# Autodesk Inventor assembly: frame
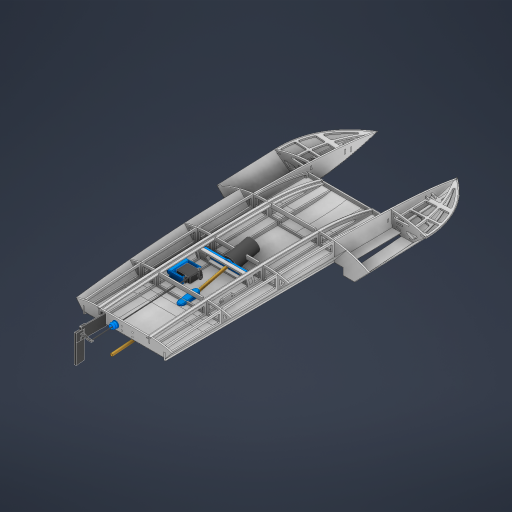
[picture p0: Inventor's stored thumbnail of the model, 512x512]
Saved by Autodesk Inventor 2023 (Build 270158030, 158C)
## iProperties
Created: 2022-03-21
Part Number: frame
Document SubType Name: Assembly
Designer: kardo
Mass: 464.87 g
Surface Area: 7011.93 cm^2
Volume: 464.87 cm^3
Density: 1 g/cm^3
Author: kardo
## Documents named in this file (42)
- D:\Computer Aided Design\hydroplane_plan_2_refactor\model\shape\frame\frame.iam
- D:\Computer Aided Design\hydroplane_plan_2_refactor\model\shape\frame\bulkheads\main.ipt
- D:\Computer Aided Design\hydroplane_plan_2_refactor\model\shape\frame\bulkheads\transom.ipt
- D:\Computer Aided Design\hydroplane_plan_2_refactor\model\shape\frame\bulkheads\stringer.ipt
- D:\Computer Aided Design\hydroplane_plan_2_refactor\model\shape\frame\bulkheads\tail_2.ipt
- D:\Computer Aided Design\hydroplane_plan_2_refactor\model\shape\frame\bulkheads\tail_1.ipt
- D:\Computer Aided Design\hydroplane_plan_2_refactor\model\shape\frame\bulkheads\sponson_break.ipt
- D:\Computer Aided Design\hydroplane_plan_2_refactor\model\shape\frame\bulkheads\nose.ipt
- D:\Computer Aided Design\hydroplane_plan_2_refactor\model\shape\frame\bulkheads\sponson_spanner_side.ipt
- D:\Computer Aided Design\hydroplane_plan_2_refactor\model\shape\frame\bulkheads\sponson_spanner_bottom.ipt
- D:\Computer Aided Design\hydroplane_plan_2_refactor\model\shape\frame\bulkheads\sponson_spanner_bottom_holder.ipt
- D:\Computer Aided Design\hydroplane_plan_2_refactor\model\shape\frame\bulkheads\sponson_spanner_side_holder.ipt
- D:\Computer Aided Design\hydroplane_plan_2_refactor\model\shape\frame\bulkheads\stringer_cowl.ipt
- D:\Computer Aided Design\hydroplane_plan_2_refactor\model\shape\frame\bulkheads\standoff.ipt
- D:\Computer Aided Design\hydroplane_plan_2_refactor\model\shape\frame\shell\bottom.ipt
- D:\Computer Aided Design\hydroplane_plan_2_refactor\model\shape\frame\mirrored\bottom_MIR.ipt
- D:\Computer Aided Design\hydroplane_plan_2_refactor\model\shape\frame\shell\bottom_standoff.ipt
- D:\Computer Aided Design\hydroplane_plan_2_refactor\model\shape\frame\shell\sponson_bottom.ipt
- D:\Computer Aided Design\hydroplane_plan_2_refactor\model\shape\frame\mirrored\sponson_bottom_MIR.ipt
- D:\Computer Aided Design\hydroplane_plan_2_refactor\model\shape\frame\shell\sponson_indent.ipt
- D:\Computer Aided Design\hydroplane_plan_2_refactor\model\shape\frame\mirrored\sponson_indent_MIR.ipt
- D:\Computer Aided Design\hydroplane_plan_2_refactor\model\shape\frame\shell\sponson_side.ipt
- D:\Computer Aided Design\hydroplane_plan_2_refactor\model\shape\frame\mirrored\sponson_side_MIR.ipt
- D:\Computer Aided Design\hydroplane_plan_2_refactor\model\shape\frame\shell\tail_side.ipt
- D:\Computer Aided Design\hydroplane_plan_2_refactor\model\shape\frame\mirrored\tail_side_MIR.ipt
- D:\Computer Aided Design\hydroplane_plan_2_refactor\model\shape\frame\shell\cowl_liner.ipt
- D:\Computer Aided Design\hydroplane_plan_2_refactor\model\shape\frame\shell\sealing_liner.ipt
- D:\Computer Aided Design\hydroplane_plan_2_refactor\model\shape\frame\bulkheads\motor_mount.ipt
- D:\Computer Aided Design\hydroplane_plan_2_refactor\model\shape\frame\plastics\shaft_outlet.ipt
- D:\Computer Aided Design\hydroplane_plan_2_refactor\model\shape\frame\plastics\servo_mount.ipt
- D:\Computer Aided Design\hydroplane_plan_2_refactor\model\shape\frame\hardware\servo.iam
- D:\Computer Aided Design\hydroplane_plan_2_refactor\model\shape\frame\hardware\rudder.iam
- D:\Computer Aided Design\hydroplane_plan_2_refactor\model\shape\frame\hardware\steering_rod.ipt
- D:\Computer Aided Design\hydroplane_plan_2_refactor\model\shape\frame\plastics\motor_mount_plate.ipt
- D:\Computer Aided Design\hydroplane_plan_2_refactor\model\shape\frame\hardware\motor.ipt
- D:\Computer Aided Design\hydroplane_plan_2_refactor\model\shape\frame\hardware\prop_shaft.ipt
- D:\Computer Aided Design\hydroplane_plan_2_refactor\model\shape\frame\shell\deck.ipt
- D:\Computer Aided Design\hydroplane_plan_2_refactor\model\shape\frame\mirrored\deck_MIR.ipt
- D:\Computer Aided Design\hydroplane_plan_2_refactor\model\shape\frame\bulkheads\nose_spanner.ipt
- D:\Computer Aided Design\hydroplane_plan_2_refactor\model\shape\frame\shell\deck_nose.ipt
- D:\Computer Aided Design\hydroplane_plan_2_refactor\model\shape\frame\mirrored\deck_nose_MIR.ipt
- D:\Computer Aided Design\hydroplane_plan_2_refactor\model\shape\frame\plastics\servo_rod_outlet.ipt
## Components (52 placed, 41 different names)
1. main:1 — Mate:47, Mate:48, Mate:49, Mate:50, Mate:51, Mate:52, Mate:53, Mate:54, Mate:55, Mate:56, Mate:57, Mate:58, Mate:67, Mate:68, Mate:69, Mate:70, Mate:71, Mate:72, Mate:73, Mate:74, Mate:75, Mate:76, Mate:77, Mate:78, Mate:79, Mate:80, Mate:81, Mate:83, Mate:85, Mate:87, Mate:89, Mate:90, Mate:91, Mate:92, Mate:93, Mate:95, Mate:96, Mate:97, Mate:99, Mate:100, Mate:101, Mate:102, Mate:123, Mate:124, Mate:125, Mate:126, Mate:127, Mate:128, Mate:135, Mate:136, Mate:137, Mate:138
2. servo_rod_outlet:1 — Mate:145, Mate:146
3. nose_spanner:2 — Mate:132, Mate:133, Mate:134
4. nose_spanner:1 — Mate:129, Mate:130, Mate:131
5. motor_mount:1 — Mate:105, Mate:106, Mate:118, Mate:119, Mate:120
6. standoff:1 — Mate:85, Mate:86, Mate:87, Mate:88
7. standoff:2 — Mate:81, Mate:82, Mate:83, Mate:84
8. transom:1 — Mate:5, Mate:6, Mate:94, Mate:98, Mate:103, Mate:104, Mate:115, Mate:116, Mate:117, Mate:145, Mate:146
9. stringer:1 — Mate:13, Mate:14, Mate:29, Mate:30, Mate:31, Mate:32, Mate:34, Mate:53, Mate:54, Mate:133
10. stringer:2 — Mate:5, Mate:6, Mate:7, Mate:8, Mate:9, Mate:10, Mate:11, Mate:12, Mate:15, Mate:16, Mate:25, Mate:26, Mate:27, Mate:28, Mate:33, Mate:51, Mate:52, Mate:130
11. tail_2:1 — Mate:7, Mate:8
12. tail_1:1 — Mate:9, Mate:10, Mate:82, Mate:86
13. sponson_break:1 — Mate:11, Mate:12, Mate:17, Mate:19, Mate:20
14. sponson_break:2 — Mate:13, Mate:14, Mate:21, Mate:23, Mate:24
15. nose:1 — Mate:15, Mate:16, Mate:84, Mate:88, Mate:129, Mate:131, Mate:132, Mate:134
16. sponson_spanner_side:1 — Mate:17, Mate:33
17. sponson_spanner_side:2 — Mate:21, Mate:34
18. sponson_spanner_bottom:1 — Mate:19, Mate:20
19. sponson_spanner_bottom:2 — Mate:23, Mate:24
20. sponson_spanner_bottom_holder:1 — Mate:25, Mate:26
21. sponson_spanner_bottom_holder:2 — Mate:29, Mate:30
22. sponson_spanner_side_holder:1 — Mate:27, Mate:28
23. sponson_spanner_side_holder:2 — Mate:31, Mate:32
24. stringer_cowl:1 — Mate:57, Mate:58, Mate:105, Mate:106
25. stringer_cowl:2 — Mate:55, Mate:56, Mate:139, Mate:140, Mate:141
26. deck_nose:1 — Mate:135, Mate:136
27. deck_nose_MIR:1 — Mate:137, Mate:138
28. deck:1 — Mate:125, Mate:126
29. deck_MIR:1 — Mate:127, Mate:128
30. cowl_liner:1 — Mate:96, Mate:97, Mate:98
31. cowl_liner:2 — Mate:93, Mate:94, Mate:95
32. sealing_liner:1 — Mate:99, Mate:102, Mate:103
33. sealing_liner:2 — Mate:100, Mate:101, Mate:104
34. tail_side:1 — Mate:89, Mate:90
35. tail_side_MIR:1 — Mate:91, Mate:92
36. sponson_side:1 — Mate:77, Mate:78
37. sponson_side_MIR:1 — Mate:79, Mate:80
38. sponson_bottom:1 — Mate:69, Mate:70
39. sponson_bottom_MIR:1 — Mate:71, Mate:72
40. sponson_indent:1 — Mate:73, Mate:74
41. sponson_indent_MIR:1 — Mate:75, Mate:76
42. bottom_standoff:1 — Mate:67, Mate:68, Mate:107, Mate:108
43. bottom:1 — Mate:47, Mate:48
44. bottom_MIR:1 — Mate:49, Mate:50
45. rudder:1 [sub-assembly] — Mate:115, Mate:116, Mate:117, Ball:1
46. steering_rod:1 — Ball:1, Ball:2
47. motor:1 — Mate:121, Mate:122
48. prop_shaft:1 — Mate:123, Mate:124
49. servo:1 [sub-assembly] — Ball:2, Mate:142, Mate:143, Mate:144
50. motor_mount_plate:1 — Mate:118, Mate:119, Mate:120, Mate:121, Mate:122
51. servo_mount:1 — Mate:139, Mate:140, Mate:141, Mate:142, Mate:143, Mate:144
52. shaft_outlet:1 — Mate:107, Mate:108
## Relationships (116: Mate 114, BallJoint 2)
- Mate:5: transom:1 ↔ stringer:2
- Mate:6: transom:1 ↔ stringer:2
- Mate:7: stringer:2 ↔ tail_2:1
- Mate:8: stringer:2 ↔ tail_2:1
- Mate:9: stringer:2 ↔ tail_1:1
- Mate:10: stringer:2 ↔ tail_1:1
- Mate:11: stringer:2 ↔ sponson_break:1
- Mate:12: stringer:2 ↔ sponson_break:1
- Mate:13: stringer:1 ↔ sponson_break:2
- Mate:14: stringer:1 ↔ sponson_break:2
- Mate:15: stringer:2 ↔ nose:1
- Mate:16: stringer:2 ↔ nose:1
- Mate:17: sponson_break:1 ↔ sponson_spanner_side:1
- Mate:19: sponson_break:1 ↔ sponson_spanner_bottom:1
- Mate:20: sponson_break:1 ↔ sponson_spanner_bottom:1
- Mate:21: sponson_break:2 ↔ sponson_spanner_side:2
- Mate:23: sponson_break:2 ↔ sponson_spanner_bottom:2
- Mate:24: sponson_break:2 ↔ sponson_spanner_bottom:2
- Mate:25: stringer:2 ↔ sponson_spanner_bottom_holder:1
- Mate:26: stringer:2 ↔ sponson_spanner_bottom_holder:1
- Mate:27: stringer:2 ↔ sponson_spanner_side_holder:1
- Mate:28: stringer:2 ↔ sponson_spanner_side_holder:1
- Mate:29: stringer:1 ↔ sponson_spanner_bottom_holder:2
- Mate:30: stringer:1 ↔ sponson_spanner_bottom_holder:2
- Mate:31: stringer:1 ↔ sponson_spanner_side_holder:2
- Mate:32: stringer:1 ↔ sponson_spanner_side_holder:2
- Mate:33: stringer:2 ↔ sponson_spanner_side:1
- Mate:34: stringer:1 ↔ sponson_spanner_side:2
- Mate:47: main:1 ↔ bottom:1
- Mate:48: main:1 ↔ bottom:1
- Mate:49: main:1 ↔ bottom_MIR:1
- Mate:50: main:1 ↔ bottom_MIR:1
- Mate:51: main:1 ↔ stringer:2
- Mate:52: main:1 ↔ stringer:2
- Mate:53: main:1 ↔ stringer:1
- Mate:54: main:1 ↔ stringer:1
- Mate:55: main:1 ↔ stringer_cowl:2
- Mate:56: main:1 ↔ stringer_cowl:2
- Mate:57: main:1 ↔ stringer_cowl:1
- Mate:58: main:1 ↔ stringer_cowl:1
- Mate:67: main:1 ↔ bottom_standoff:1
- Mate:68: main:1 ↔ bottom_standoff:1
- Mate:69: main:1 ↔ sponson_bottom:1
- Mate:70: main:1 ↔ sponson_bottom:1
- Mate:71: main:1 ↔ sponson_bottom_MIR:1
- Mate:72: main:1 ↔ sponson_bottom_MIR:1
- Mate:73: main:1 ↔ sponson_indent:1
- Mate:74: main:1 ↔ sponson_indent:1
- Mate:75: main:1 ↔ sponson_indent_MIR:1
- Mate:76: main:1 ↔ sponson_indent_MIR:1
- Mate:77: main:1 ↔ sponson_side:1
- Mate:78: main:1 ↔ sponson_side:1
- Mate:79: main:1 ↔ sponson_side_MIR:1
- Mate:80: main:1 ↔ sponson_side_MIR:1
- Mate:81: main:1 ↔ standoff:2
- Mate:82: standoff:2 ↔ tail_1:1
- Mate:83: main:1 ↔ standoff:2
- Mate:84: standoff:2 ↔ nose:1
- Mate:85: main:1 ↔ standoff:1
- Mate:86: standoff:1 ↔ tail_1:1
- Mate:87: main:1 ↔ standoff:1
- Mate:88: standoff:1 ↔ nose:1
- Mate:89: main:1 ↔ tail_side:1
- Mate:90: main:1 ↔ tail_side:1
- Mate:91: main:1 ↔ tail_side_MIR:1
- Mate:92: main:1 ↔ tail_side_MIR:1
- Mate:93: main:1 ↔ cowl_liner:2
- Mate:94: transom:1 ↔ cowl_liner:2
- Mate:95: main:1 ↔ cowl_liner:2
- Mate:96: main:1 ↔ cowl_liner:1
- Mate:97: main:1 ↔ cowl_liner:1
- Mate:98: transom:1 ↔ cowl_liner:1
- Mate:99: main:1 ↔ sealing_liner:1
- Mate:100: main:1 ↔ sealing_liner:2
- Mate:101: main:1 ↔ sealing_liner:2
- Mate:102: main:1 ↔ sealing_liner:1
- Mate:103: transom:1 ↔ sealing_liner:1
- Mate:104: transom:1 ↔ sealing_liner:2
- Mate:105: motor_mount:1 ↔ stringer_cowl:1
- Mate:106: motor_mount:1 ↔ stringer_cowl:1
- Mate:107: bottom_standoff:1 ↔ shaft_outlet:1
- Mate:108: bottom_standoff:1 ↔ shaft_outlet:1
- Mate:115: transom:1 ↔ rudder:1
- Mate:116: transom:1 ↔ rudder:1
- Mate:117: transom:1 ↔ rudder:1
- Ball:1: rudder:1 ↔ steering_rod:1
- Ball:2: steering_rod:1 ↔ servo:1
- Mate:118: motor_mount:1 ↔ motor_mount_plate:1
- Mate:119: motor_mount:1 ↔ motor_mount_plate:1
- Mate:120: motor_mount:1 ↔ motor_mount_plate:1
- Mate:121: motor:1 ↔ motor_mount_plate:1
- Mate:122: motor:1 ↔ motor_mount_plate:1
- Mate:123: main:1 ↔ prop_shaft:1
- Mate:124: main:1 ↔ prop_shaft:1
- Mate:125: main:1 ↔ deck:1
- Mate:126: main:1 ↔ deck:1
- Mate:127: main:1 ↔ deck_MIR:1
- Mate:128: main:1 ↔ deck_MIR:1
- Mate:129: nose_spanner:1 ↔ nose:1
- Mate:130: nose_spanner:1 ↔ stringer:2
- Mate:131: nose_spanner:1 ↔ nose:1
- Mate:132: nose_spanner:2 ↔ nose:1
- Mate:133: nose_spanner:2 ↔ stringer:1
- Mate:134: nose_spanner:2 ↔ nose:1
- Mate:135: main:1 ↔ deck_nose:1
- Mate:136: main:1 ↔ deck_nose:1
- Mate:137: main:1 ↔ deck_nose_MIR:1
- Mate:138: main:1 ↔ deck_nose_MIR:1
- Mate:139: stringer_cowl:2 ↔ servo_mount:1
- Mate:140: stringer_cowl:2 ↔ servo_mount:1
- Mate:141: stringer_cowl:2 ↔ servo_mount:1
- Mate:142: servo:1 ↔ servo_mount:1
- Mate:143: servo:1 ↔ servo_mount:1
- Mate:144: servo:1 ↔ servo_mount:1
- Mate:145: servo_rod_outlet:1 ↔ transom:1
- Mate:146: servo_rod_outlet:1 ↔ transom:1
